# Autodesk Inventor assembly: CAD FINAL DELIVERABLE
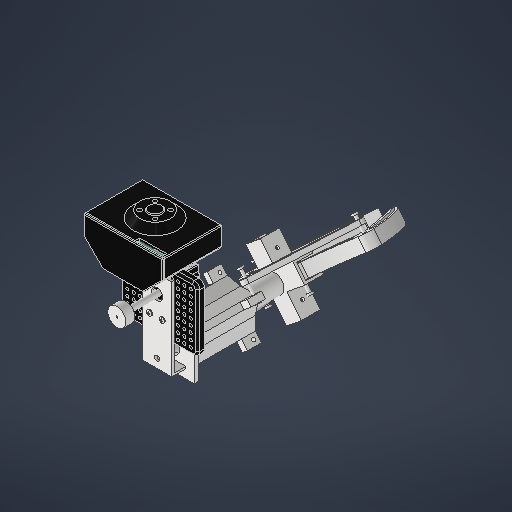
[picture p0: Inventor's stored thumbnail of the model, 512x512]
Saved by Autodesk Inventor 2026 (Build 300175050, 175E)
## iProperties
Created: 2025-11-30
Part Number: CAD FINAL DELIVERABLE
Document SubType Name: Assembly
Designer: sarab
Author: sarab
## Documents named in this file (14)
- C:\Users\exp-213\Desktop\FINAL ASSEMBLY FILE\CAD FINAL DELIVERABLE.iam
- C:\Users\exp-213\Desktop\FINAL ASSEMBLY FILE\End Effector Platform.iam
- C:\Users\exp-213\Desktop\FINAL ASSEMBLY FILE\Top Connecter 1.ipt
- C:\Users\exp-213\Desktop\FINAL ASSEMBLY FILE\Top Connecter 2.ipt
- C:\Users\exp-213\Desktop\FINAL ASSEMBLY FILE\Lifter compartment.ipt
- C:\Users\exp-213\Desktop\FINAL ASSEMBLY FILE\Lifter.ipt
- C:\Users\exp-213\Desktop\FINAL ASSEMBLY FILE\Lifter Connecter.ipt
- C:\Users\exp-213\Desktop\FINAL ASSEMBLY FILE\Screw.ipt
- C:\Users\exp-213\Desktop\FINAL ASSEMBLY FILE\Bracket.ipt
- C:\Users\exp-213\Desktop\FINAL ASSEMBLY FILE\Claw.ipt
- C:\Users\exp-213\Desktop\FINAL ASSEMBLY FILE\Screw cap.ipt
- C:\Users\exp-213\Desktop\FINAL ASSEMBLY FILE\string holder.iam
- C:\Users\exp-213\Desktop\FINAL ASSEMBLY FILE\Fasteners\Steel M3 Hex Nut.ipt
- C:\Users\exp-213\Desktop\FINAL ASSEMBLY FILE\Fasteners\Steel M3x16 Pan Head Screw.ipt
## Components (27 placed, 13 different names)
1. End Effector Platform:1 [sub-assembly] — Insert:1, Mate:1, Angle:1, Insert:2, Angle:2, Angle:3, Insert:29, Insert:30
2. string holder:1 [sub-assembly] — Insert:1, Rotation/Translation:1
3. Top Connecter 1:1 — Mate:1, Angle:1, Insert:2, Mate:2, Angle:9, Angle:10, Angle:12, Angle:13, Angle:14, Angle:15, Angle:16, Insert:27, Insert:28
4. Top Connecter 2:1 — Mate:2, Mate:3, Insert:3, Angle:5, Angle:6, Angle:7, Angle:8, Angle:11, Angle:17, Angle:18, Angle:19, Angle:20
5. Lifter compartment:1 — Mate:3, Angle:2, Insert:3, Insert:4, Flush:5, Flush:6, Insert:5, Insert:6, Insert:12, Insert:20
6. Lifter:1 — Insert:4, Angle:3, Mate:4, Flush:2, Flush:4, Rotation/Translation:1
7. Lifter Connecter:1 — Mate:4, Flush:5, Flush:6, Insert:11, Insert:17, Insert:19, Insert:25
8. Bracket:1 — Insert:5, Insert:23
9. Bracket:2 — Insert:6, Insert:14
10. Screw:1 — Insert:12, Insert:13, Angle:7
11. Screw:2 — Angle:5, Insert:20, Insert:21
12. Screw cap:1 — Angle:6, Insert:21
13. Screw cap:2 — Insert:13, Angle:8
14. Claw:1 — Insert:11, Insert:14, Insert:15
15. Claw:2 — Insert:19, Insert:22, Insert:23
16. Screw:3 — Insert:15, Insert:16, Angle:10
17. Screw:4 — Insert:17, Insert:18, Angle:12
18. Screw cap:3 — Insert:16, Angle:9
19. Screw cap:4 — Insert:18, Angle:11
20. Screw:5 — Insert:22, Angle:13, Insert:24
21. Screw:6 — Insert:25, Angle:15, Insert:26
22. Screw cap:5 — Insert:24, Angle:14
23. Screw cap:6 — Insert:26, Angle:16
24. Steel M3 Hex Nut:1 — Insert:30, Angle:17
25. Steel M3 Hex Nut:2 — Insert:29, Angle:18
26. Steel M3x16 Pan Head Screw:1 — Insert:28, Angle:20
27. Steel M3x16 Pan Head Screw:2 — Insert:27, Angle:19
## Relationships (54: Insert 26, Angle 19, Mate 4, Flush 4, RelateRotateTranslate 1)
- Insert:1: End Effector Platform:1 ↔ string holder:1
- Mate:1: End Effector Platform:1 ↔ Top Connecter 1:1
- Angle:1 (0 deg): End Effector Platform:1 ↔ Top Connecter 1:1
- Insert:2: End Effector Platform:1 ↔ Top Connecter 1:1
- Mate:2: Top Connecter 1:1 ↔ Top Connecter 2:1
- Mate:3: Top Connecter 2:1 ↔ Lifter compartment:1
- Angle:2 (0 deg): End Effector Platform:1 ↔ Lifter compartment:1
- Insert:3: Top Connecter 2:1 ↔ Lifter compartment:1
- Insert:4: Lifter compartment:1 ↔ Lifter:1
- Angle:3 (0 deg): End Effector Platform:1 ↔ Lifter:1
- Mate:4: Lifter:1 ↔ Lifter Connecter:1
- Flush:2: Lifter:1
- Flush:4: Lifter:1
- Flush:5: Lifter compartment:1 ↔ Lifter Connecter:1
- Flush:6: Lifter compartment:1 ↔ Lifter Connecter:1
- Insert:5: Lifter compartment:1 ↔ Bracket:1
- Insert:6: Lifter compartment:1 ↔ Bracket:2
- Angle:5 (0 deg): Top Connecter 2:1 ↔ Screw:2
- Angle:6 (0 deg): Top Connecter 2:1 ↔ Screw cap:1
- Insert:11: Lifter Connecter:1 ↔ Claw:1
- Insert:12: Lifter compartment:1 ↔ Screw:1
- Insert:13: Screw:1 ↔ Screw cap:2
- Angle:7 (0 deg): Top Connecter 2:1 ↔ Screw:1
- Angle:8 (0 deg): Top Connecter 2:1 ↔ Screw cap:2
- Insert:14: Bracket:2 ↔ Claw:1
- Insert:15: Claw:1 ↔ Screw:3
- Insert:16: Screw:3 ↔ Screw cap:3
- Angle:9 (0 deg): Top Connecter 1:1 ↔ Screw cap:3
- Angle:10 (0 deg): Top Connecter 1:1 ↔ Screw:3
- Insert:17: Lifter Connecter:1 ↔ Screw:4
- Insert:18: Screw:4 ↔ Screw cap:4
- Angle:11 (0 deg): Top Connecter 2:1 ↔ Screw cap:4
- Angle:12 (0 deg): Top Connecter 1:1 ↔ Screw:4
- Insert:19: Lifter Connecter:1 ↔ Claw:2
- Insert:20: Lifter compartment:1 ↔ Screw:2
- Insert:21: Screw:2 ↔ Screw cap:1
- Insert:22: Claw:2 ↔ Screw:5
- Angle:13 (0 deg): Top Connecter 1:1 ↔ Screw:5
- Insert:23: Bracket:1 ↔ Claw:2
- Insert:24: Screw:5 ↔ Screw cap:5
- Angle:14 (0 deg): Top Connecter 1:1 ↔ Screw cap:5
- Insert:25: Lifter Connecter:1 ↔ Screw:6
- Angle:15 (0 deg): Top Connecter 1:1 ↔ Screw:6
- Insert:26: Screw:6 ↔ Screw cap:6
- Angle:16 (0 deg): Top Connecter 1:1 ↔ Screw cap:6
- Rotation/Translation:1 [RelateRotateTranslate] (18.85 mm): string holder:1 ↔ Lifter:1
- Insert:27: Top Connecter 1:1 ↔ Steel M3x16 Pan Head Screw:2
- Insert:28: Top Connecter 1:1 ↔ Steel M3x16 Pan Head Screw:1
- Insert:29: End Effector Platform:1 ↔ Steel M3 Hex Nut:2
- Insert:30: End Effector Platform:1 ↔ Steel M3 Hex Nut:1
- Angle:17 (0 deg): Top Connecter 2:1 ↔ Steel M3 Hex Nut:1
- Angle:18 (0 deg): Top Connecter 2:1 ↔ Steel M3 Hex Nut:2
- Angle:19 (0 deg): Top Connecter 2:1 ↔ Steel M3x16 Pan Head Screw:2
- Angle:20 (0 deg): Top Connecter 2:1 ↔ Steel M3x16 Pan Head Screw:1
